# Autodesk Inventor assembly: クランク_MIR
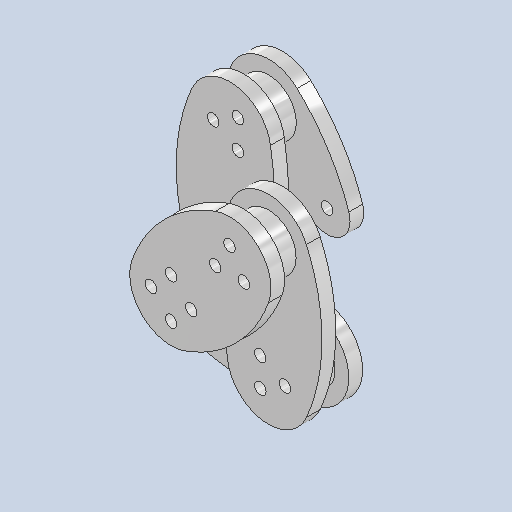
[picture p0: Inventor's stored thumbnail of the model, 512x512]
Saved by Autodesk Inventor 2023 (Build 270158000, 158)
## iProperties
Created: 2022-01-08
Part Number: クランク_MIR
Document SubType Name: Assembly
Designer: muzho
Author: acps
## Documents named in this file (5)
- C:\Users\muzho\Documents\srdc\srdc_2\脚\ミラー\クランク_MIR.iam
- C:\Users\muzho\Documents\srdc\srdc_2\脚\ミラー\カム3_MIR.ipt
- C:\Users\muzho\Documents\srdc\srdc_2\脚\ミラー\クランク_前_MIR.ipt
- C:\Users\muzho\Documents\srdc\srdc_2\脚\ミラー\クランク_中間_MIR.ipt
- C:\Users\muzho\Documents\srdc\srdc_2\脚\ミラー\駆動節_MIR.ipt
## Components (9 placed, 4 different names)
1. カム3_MIR:1 — 挿入:9, メイト:18, メイト:17, 挿入:2, メイト:4, メイト:3
2. カム3_MIR:2 — 挿入:3, メイト:6, メイト:5, 挿入:4, メイト:8, メイト:7
3. カム3_MIR:3 — 挿入:10, メイト:10, メイト:9, 挿入:6, メイト:12, メイト:11
4. クランク_前_MIR:1 — 挿入:9, メイト:18, メイト:17
5. クランク_中間_MIR:1 — 挿入:3, メイト:6, メイト:5, 挿入:2, メイト:4, メイト:3
6. クランク_中間_MIR:2 — 挿入:10, メイト:10, メイト:9, 挿入:4, メイト:8, メイト:7
7. クランク_中間_MIR:3 — 挿入:6, メイト:12, メイト:11, 挿入:7, メイト:14, メイト:13
8. カム3_MIR:4 — 挿入:7, メイト:14, メイト:13, 挿入:8, メイト:16, メイト:15
9. 駆動節_MIR:1 — 挿入:8, メイト:16, メイト:15
## Relationships (24: Mate 16, Insert 8)
- 挿入:9 [Insert]: カム3_MIR:1 ↔ クランク_前_MIR:1
- メイト:18 [Mate]: カム3_MIR:1 ↔ クランク_前_MIR:1
- メイト:17 [Mate]: カム3_MIR:1 ↔ クランク_前_MIR:1
- 挿入:3 [Insert]: カム3_MIR:2 ↔ クランク_中間_MIR:1
- メイト:6 [Mate]: カム3_MIR:2 ↔ クランク_中間_MIR:1
- メイト:5 [Mate]: カム3_MIR:2 ↔ クランク_中間_MIR:1
- 挿入:2 [Insert]: カム3_MIR:1 ↔ クランク_中間_MIR:1
- メイト:4 [Mate]: カム3_MIR:1 ↔ クランク_中間_MIR:1
- メイト:3 [Mate]: カム3_MIR:1 ↔ クランク_中間_MIR:1
- 挿入:10 [Insert]: カム3_MIR:3 ↔ クランク_中間_MIR:2
- メイト:10 [Mate]: カム3_MIR:3 ↔ クランク_中間_MIR:2
- メイト:9 [Mate]: カム3_MIR:3 ↔ クランク_中間_MIR:2
- 挿入:4 [Insert]: カム3_MIR:2 ↔ クランク_中間_MIR:2
- メイト:8 [Mate]: カム3_MIR:2 ↔ クランク_中間_MIR:2
- メイト:7 [Mate]: カム3_MIR:2 ↔ クランク_中間_MIR:2
- 挿入:6 [Insert]: カム3_MIR:3 ↔ クランク_中間_MIR:3
- メイト:12 [Mate]: カム3_MIR:3 ↔ クランク_中間_MIR:3
- メイト:11 [Mate]: カム3_MIR:3 ↔ クランク_中間_MIR:3
- 挿入:7 [Insert]: クランク_中間_MIR:3 ↔ カム3_MIR:4
- メイト:14 [Mate]: クランク_中間_MIR:3 ↔ カム3_MIR:4
- メイト:13 [Mate]: クランク_中間_MIR:3 ↔ カム3_MIR:4
- 挿入:8 [Insert]: カム3_MIR:4 ↔ 駆動節_MIR:1
- メイト:16 [Mate]: カム3_MIR:4 ↔ 駆動節_MIR:1
- メイト:15 [Mate]: カム3_MIR:4 ↔ 駆動節_MIR:1
